# Autodesk Inventor assembly: Montagemsemfuros
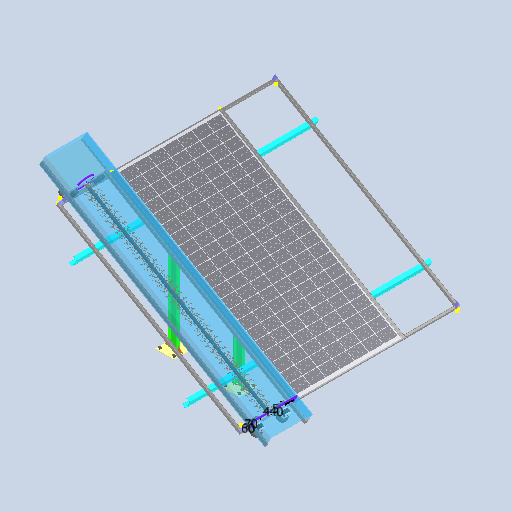
[picture p0: Inventor's stored thumbnail of the model, 512x512]
Saved by Autodesk Inventor 2025.3 (Build 293356030, 356C)
## iProperties
Created: 2019-12-15
Part Number: Montagemsemfuros
Document SubType Name: Assembly
Designer: Rubens
Sending System: SolidWorks 2021
Last Author: Mohsen
Last Saved: 2022-08-25
Author: Rubens
## Documents named in this file (36)
- C:\Users\Rubens\Downloads\Estrutura Placa - REV00\Solar Mounting Structure\Main_Solar_Structure\Main_Solar_Structure\Montagemsemfuros.iam
- C:\Users\Rubens\Downloads\Estrutura Placa - REV00\Solar Mounting Structure\Main_Solar_Structure\Main_Solar_Structure\Small_Column.ipt
- C:\Users\Rubens\Downloads\Estrutura Placa - REV00\Solar Mounting Structure\Main_Solar_Structure\Main_Solar_Structure\Large_Column.ipt
- C:\Users\Rubens\Downloads\Estrutura Placa - REV00\Solar Mounting Structure\Main_Solar_Structure\Main_Solar_Structure\Bottom_Beam.ipt
- C:\Users\Rubens\Downloads\Estrutura Placa - REV00\Solar Mounting Structure\Main_Solar_Structure\Main_Solar_Structure\Base_Plate.ipt
- C:\Users\Rubens\Downloads\Estrutura Placa - REV00\Solar Mounting Structure\Main_Solar_Structure\Main_Solar_Structure\Base_Support.ipt
- C:\Users\Rubens\Downloads\Estrutura Placa - REV00\Solar Mounting Structure\Main_Solar_Structure\Main_Solar_Structure\Beam_Support.ipt
- C:\Users\Rubens\Downloads\Estrutura Placa - REV00\Solar Mounting Structure\Main_Solar_Structure\Main_Solar_Structure\M10_Screw&Nut.iam
- C:\Users\Rubens\Downloads\Estrutura Placa - REV00\Solar Mounting Structure\Main_Solar_Structure\Main_Solar_Structure\Base.ipt
- C:\Users\Rubens\Downloads\Estrutura Placa - REV00\Solar Mounting Structure\Main_Solar_Structure\Main_Solar_Structure\ISO - 4034 - M16 - S_.ipt
- C:\Users\Rubens\Downloads\Estrutura Placa - REV00\Solar Mounting Structure\Main_Solar_Structure\Main_Solar_Structure\Base_MIR.ipt
- C:\Users\Rubens\Downloads\Estrutura Placa - REV00\Solar Mounting Structure\Main_Solar_Structure\Main_Solar_Structure\Base_Plate_MIR.ipt
- C:\Users\Rubens\Downloads\Estrutura Placa - REV00\Solar Mounting Structure\Main_Solar_Structure\Main_Solar_Structure\Base_Support_MIR.ipt
- C:\Users\Rubens\Downloads\Estrutura Placa - REV00\Solar Mounting Structure\Main_Solar_Structure\Main_Solar_Structure\Base_MIR1.ipt
- C:\Users\Rubens\Downloads\Estrutura Placa - REV00\Solar Mounting Structure\Main_Solar_Structure\Main_Solar_Structure\ISO - 4034 - M16 - S__MIR.ipt
- C:\Users\Rubens\Downloads\Estrutura Placa - REV00\Solar Mounting Structure\Main_Solar_Structure\Main_Solar_Structure\Base_MIR_MIR.ipt
- C:\Users\Rubens\Downloads\Estrutura Placa - REV00\Solar Mounting Structure\Main_Solar_Structure\Main_Solar_Structure\Top_Beam_2780.ipt
- C:\Users\Rubens\Downloads\Estrutura Placa - REV00\Solar Mounting Structure\Main_Solar_Structure\Main_Solar_Structure\Beam_Support_MIR.ipt
- C:\Users\Rubens\Downloads\Estrutura Placa - REV00\Solar Mounting Structure\Main_Solar_Structure\Main_Solar_Structure\SolarPV.ipt
- C:\Users\Rubens\Downloads\Estrutura Placa - REV00\Solar Mounting Structure\Main_Solar_Structure\Main_Solar_Structure\Perfil tubo - 30x30x3.ipt
- C:\Users\Rubens\Downloads\Estrutura Placa - REV00\Solar Mounting Structure\Main_Solar_Structure\Main_Solar_Structure\tubo 30 x 30 x 3  - 500.ipt
- C:\Users\Rubens\Downloads\Estrutura Placa - REV00\Solar Mounting Structure\Main_Solar_Structure\Main_Solar_Structure\Limitador.ipt
- C:\Users\Rubens\Downloads\Estrutura Placa - REV00\Solar Mounting Structure\Main_Solar_Structure\Main_Solar_Structure\Small_Column_MIR2.ipt
- C:\Users\Rubens\Downloads\Estrutura Placa - REV00\Solar Mounting Structure\Main_Solar_Structure\Main_Solar_Structure\Bottom_Beam_MIR2.ipt
- C:\Users\Rubens\Downloads\Estrutura Placa - REV00\Solar Mounting Structure\Main_Solar_Structure\Main_Solar_Structure\Base_Plate_MIR3.ipt
- C:\Users\Rubens\Downloads\Estrutura Placa - REV00\Solar Mounting Structure\Main_Solar_Structure\Main_Solar_Structure\Base_Support_MIR3.ipt
- C:\Users\Rubens\Downloads\Estrutura Placa - REV00\Solar Mounting Structure\Main_Solar_Structure\Main_Solar_Structure\M10_Screw&Nut_MIR1.iam
- C:\Users\Rubens\Downloads\Estrutura Placa - REV00\Solar Mounting Structure\Main_Solar_Structure\Main_Solar_Structure\ISO - 4034 - M16 - S__MIR1.ipt
- C:\Users\Rubens\Downloads\Estrutura Placa - REV00\Solar Mounting Structure\Main_Solar_Structure\Main_Solar_Structure\Base_Plate_MIR_MIR2.ipt
- C:\Users\Rubens\Downloads\Estrutura Placa - REV00\Solar Mounting Structure\Main_Solar_Structure\Main_Solar_Structure\Base_Support_MIR_MIR1.ipt
- C:\Users\Rubens\Downloads\Estrutura Placa - REV00\Solar Mounting Structure\Main_Solar_Structure\Main_Solar_Structure\ISO - 4034 - M16 - S__MIR_MIR1.ipt
- C:\Users\Rubens\Downloads\Estrutura Placa - REV00\Solar Mounting Structure\Main_Solar_Structure\Main_Solar_Structure\Large_Column_MIR3.ipt
- C:\Users\Rubens\Documents\Inventor\Content Center Files\R2025\pt-BR\ANSI B18.3.1M(5)\ANSI B18.3.1M - M8x1,25 x 20(3).ipt
- C:\Users\Rubens\Documents\Inventor\Content Center Files\R2025\pt-BR\ISO 4032(2)\ISO 4032 - M8 - ISO.ipt
- C:\Users\Rubens\Documents\Inventor\Content Center Files\R2025\pt-BR\ANSI B18.3.1M(6)\ANSI B18.3.1M - M8x1,25 x 40(1).ipt
- C:\Users\Rubens\Downloads\Limpador\MontagemREV0.iam
## Components (92 placed, 35 different names)
1. Small_Column:1 — Alinhado:6, Coincidente:67
2. Bottom_Beam:1 — Coincidente:3, Coincidente:5, Coincidente:6, Coincidente:8, Coincidente:20, Coincidente:21, Coincidente:66, Alinhado:15, Coincidente:72, Ângulo:1
3. Base_Plate:1 — Alinhado:14
4. Base_Support:1
5. Base_Support:2
6. Base_Support:3
7. Beam_Support:3 — Coincidente:3, Coincidente:5, Coincidente:23
8. Beam_Support:4 — Coincidente:6, Coincidente:8, Coincidente:22
9. M10_Screw&Nut:2 [sub-assembly]
10. M10_Screw&Nut:7 [sub-assembly]
11. M10_Screw&Nut:8 [sub-assembly]
12. M10_Screw&Nut:9 [sub-assembly]
13. M10_Screw&Nut:90 [sub-assembly]
14. M10_Screw&Nut:91 [sub-assembly]
15. Base:2
16. ISO - 4034 - M16 - S_:43
17. ISO - 4034 - M16 - S_:47
18. ISO - 4034 - M16 - S_:51
19. ISO - 4034 - M16 - S_:55
20. Base_MIR:1
21. Base_Plate_MIR:1 — Alinhado:14, Coincidente:65
22. Base_Support_MIR:1
23. Base_Support_MIR:2
24. Base_Support_MIR:3
25. Base_MIR1:1
26. ISO - 4034 - M16 - S__MIR:1
27. ISO - 4034 - M16 - S__MIR:2
28. ISO - 4034 - M16 - S__MIR:3
29. Base_MIR_MIR:1
30. Top_Beam_2780:1 — Coincidente:21, Coincidente:22, Alinhado:7, Coincidente:46, Coincidente:47, Coincidente:70, Alinhado:15, Coincidente:104
31. Top_Beam_2780:2 — Coincidente:20, Coincidente:23, Alinhado:7, Coincidente:24
32. Beam_Support_MIR:1
33. Beam_Support_MIR:2 — Coincidente:70
34. SolarPV:1 — Coincidente:24, Coincidente:48, Coincidente:49, Coincidente:50, Coincidente:55, Alinhado:22, Coincidente:113
35. Perfil tubo - 30x30x3:1 — Coincidente:46, Coincidente:48, Coincidente:52, Coincidente:53, Alinhado:9, Alinhado:10, Coincidente:55, Coincidente:57, Alinhado:12, Coincidente:108, Coincidente:109, Coincidente:110, Coincidente:111, Coincidente:114
36. Perfil tubo - 30x30x3:2 — Coincidente:47, Coincidente:54, Alinhado:11, Coincidente:56, Coincidente:105, Coincidente:106, Coincidente:107
37. Perfil tubo - 30x30x3:3 — Coincidente:49, Coincidente:50, Coincidente:79, Alinhado:20, Alinhado:21, Alinhado:22, Alinhado:23
38. tubo 30 x 30 x 3  - 500:1 — Coincidente:53, Alinhado:9, Alinhado:10, Coincidente:54, Alinhado:11, Coincidente:56, Coincidente:82, Alinhado:26
39. tubo 30 x 30 x 3  - 500:2 — Coincidente:52, Coincidente:57, Alinhado:12, Coincidente:81, Coincidente:112, Alinhado:27
40. Perfil tubo - 30x30x3:4 — Coincidente:58, Alinhado:13, Coincidente:59, Coincidente:80, Coincidente:83, Alinhado:19, Coincidente:84, Coincidente:85, Coincidente:100, Coincidente:101
41. tubo 30 x 30 x 3  - 500:3 — Coincidente:58, Alinhado:13, Coincidente:59, Alinhado:21
42. tubo 30 x 30 x 3  - 500:4 — Coincidente:79, Coincidente:80, Alinhado:19, Alinhado:20, Alinhado:23
43. ISO - 4034 - M16 - S__MIR:4 — Coincidente:65
44. Large_Column:1 — Coincidente:66, Coincidente:67, Coincidente:86, Coincidente:87, Coincidente:88, Coincidente:89
45. Limitador:1 — Coincidente:83
46. Limitador:2 — Coincidente:81
47. Limitador:3 — Coincidente:82
48. Limitador:4 — Coincidente:84, Coincidente:85
49. M10_Screw&Nut:92 [sub-assembly] — Coincidente:86
50. M10_Screw&Nut:93 [sub-assembly] — Coincidente:88
51. M10_Screw&Nut:94 [sub-assembly] — Coincidente:89
52. M10_Screw&Nut:96 [sub-assembly] — Coincidente:87
53. Small_Column_MIR2:1 — Alinhado:24, Coincidente:91
54. Bottom_Beam_MIR2:1 — Coincidente:92, Ângulo:2, Coincidente:93
55. Base_Plate_MIR3:1 — Alinhado:25
56. Base_Support_MIR3:1
57. Base_Support_MIR3:2
58. Base_Support_MIR3:3
59. M10_Screw&Nut_MIR1:1 [sub-assembly]
60. M10_Screw&Nut_MIR1:2 [sub-assembly]
61. M10_Screw&Nut_MIR1:3 [sub-assembly]
62. M10_Screw&Nut_MIR1:4 [sub-assembly]
63. ISO - 4034 - M16 - S__MIR1:1
64. ISO - 4034 - M16 - S__MIR1:2
65. ISO - 4034 - M16 - S__MIR1:3
66. ISO - 4034 - M16 - S__MIR1:4
67. Base_Plate_MIR_MIR2:1 — Alinhado:25, Coincidente:90
68. Base_Support_MIR_MIR1:1
69. Base_Support_MIR_MIR1:2
70. Base_Support_MIR_MIR1:3
71. ISO - 4034 - M16 - S__MIR_MIR1:1
72. ISO - 4034 - M16 - S__MIR_MIR1:2
73. ISO - 4034 - M16 - S__MIR_MIR1:3
74. ISO - 4034 - M16 - S__MIR_MIR1:4 — Coincidente:90
75. Large_Column_MIR3:1 — Coincidente:91, Coincidente:92, Coincidente:94, Coincidente:95, Coincidente:96, Coincidente:97
76. M10_Screw&Nut_MIR1:5 [sub-assembly] — Coincidente:94
77. M10_Screw&Nut_MIR1:6 [sub-assembly] — Coincidente:95
78. M10_Screw&Nut_MIR1:7 [sub-assembly] — Coincidente:96
79. M10_Screw&Nut_MIR1:8 [sub-assembly] — Coincidente:97
80. Parafuso Allen de cabeça forjada e furada - 6 furos - Métrica M8x1,25 x 20:1
81. ISO 4032 M8:1 — Coincidente:100
82. ISO 4032 M8:2 — Coincidente:101
83. Parafuso Allen de cabeça forjado - Métrica M8x1,25 x 40:3 — Coincidente:106
84. ISO 4032 M8:3 — Coincidente:107
85. Parafuso Allen de cabeça forjado - Métrica M8x1,25 x 40:4 — Coincidente:104
86. ISO 4032 M8:4 — Coincidente:105
87. Parafuso Allen de cabeça forjado - Métrica M8x1,25 x 40:5 — Coincidente:108
88. Parafuso Allen de cabeça forjado - Métrica M8x1,25 x 40:6 — Coincidente:109
89. ISO 4032 M8:5 — Coincidente:110
90. ISO 4032 M8:6 — Coincidente:111
91. MontagemREV0:2 [sub-assembly] — Coincidente:112, Alinhado:26, Coincidente:113
92. SolarPV:2 — Alinhado:27, Coincidente:114
## Relationships (82: Mate 61, Flush 19, Angle 2)
- Coincidente:3 [Mate]: Bottom_Beam:1 ↔ Beam_Support:3
- Coincidente:5 [Mate]: Bottom_Beam:1 ↔ Beam_Support:3
- Coincidente:6 [Mate]: Bottom_Beam:1 ↔ Beam_Support:4
- Coincidente:8 [Mate]: Bottom_Beam:1 ↔ Beam_Support:4
- Alinhado:6 [Flush] (300 mm): Small_Column:1
- Coincidente:20 [Mate]: Bottom_Beam:1 ↔ Top_Beam_2780:2
- Coincidente:21 [Mate]: Bottom_Beam:1 ↔ Top_Beam_2780:1
- Coincidente:22 [Mate]: Beam_Support:4 ↔ Top_Beam_2780:1
- Coincidente:23 [Mate]: Beam_Support:3 ↔ Top_Beam_2780:2
- Alinhado:7 [Flush]: Top_Beam_2780:1 ↔ Top_Beam_2780:2
- Coincidente:24 [Mate]: Top_Beam_2780:2 ↔ SolarPV:1
- Coincidente:46 [Mate]: Top_Beam_2780:1 ↔ Perfil tubo - 30x30x3:1
- Coincidente:47 [Mate]: Top_Beam_2780:1 ↔ Perfil tubo - 30x30x3:2
- Coincidente:48 [Mate]: SolarPV:1 ↔ Perfil tubo - 30x30x3:1
- Coincidente:49 [Mate]: SolarPV:1 ↔ Perfil tubo - 30x30x3:3
- Coincidente:50 [Mate]: SolarPV:1 ↔ Perfil tubo - 30x30x3:3
- Coincidente:52 [Mate]: Perfil tubo - 30x30x3:1 ↔ tubo 30 x 30 x 3  - 500:2
- Coincidente:53 [Mate]: Perfil tubo - 30x30x3:1 ↔ tubo 30 x 30 x 3  - 500:1
- Alinhado:9 [Flush]: Perfil tubo - 30x30x3:1 ↔ tubo 30 x 30 x 3  - 500:1
- Alinhado:10 [Flush]: Perfil tubo - 30x30x3:1 ↔ tubo 30 x 30 x 3  - 500:1
- Coincidente:54 [Mate]: Perfil tubo - 30x30x3:2 ↔ tubo 30 x 30 x 3  - 500:1
- Alinhado:11 [Flush]: Perfil tubo - 30x30x3:2 ↔ tubo 30 x 30 x 3  - 500:1
- Coincidente:55 [Mate]: SolarPV:1 ↔ Perfil tubo - 30x30x3:1
- Coincidente:56 [Mate]: Perfil tubo - 30x30x3:2 ↔ tubo 30 x 30 x 3  - 500:1
- Coincidente:57 [Mate]: Perfil tubo - 30x30x3:1 ↔ tubo 30 x 30 x 3  - 500:2
- Alinhado:12 [Flush]: Perfil tubo - 30x30x3:1 ↔ tubo 30 x 30 x 3  - 500:2
- Coincidente:58 [Mate]: Perfil tubo - 30x30x3:4 ↔ tubo 30 x 30 x 3  - 500:3
- Alinhado:13 [Flush]: Perfil tubo - 30x30x3:4 ↔ tubo 30 x 30 x 3  - 500:3
- Coincidente:59 [Mate]: Perfil tubo - 30x30x3:4 ↔ tubo 30 x 30 x 3  - 500:3
- Alinhado:14 [Flush]: Base_Plate:1 ↔ Base_Plate_MIR:1
- Coincidente:65 [Mate]: Base_Plate_MIR:1 ↔ ISO - 4034 - M16 - S__MIR:4
- Coincidente:66 [Mate]: Bottom_Beam:1 ↔ Large_Column:1
- Coincidente:67 [Mate] (600 mm): Small_Column:1 ↔ Large_Column:1
- Coincidente:70 [Mate]: Top_Beam_2780:1 ↔ Beam_Support_MIR:2
- Alinhado:15 [Flush] (-900 mm): Bottom_Beam:1 ↔ Top_Beam_2780:1
- Coincidente:72 [Mate]: Bottom_Beam:1
- Ângulo:1 [Angle] (0 deg): Bottom_Beam:1
- Alinhado:16 [Flush] (-450 mm)
- Coincidente:79 [Mate]: Perfil tubo - 30x30x3:3 ↔ tubo 30 x 30 x 3  - 500:4
- Coincidente:80 [Mate]: Perfil tubo - 30x30x3:4 ↔ tubo 30 x 30 x 3  - 500:4
- Coincidente:81 [Mate]: tubo 30 x 30 x 3  - 500:2 ↔ Limitador:2
- Coincidente:82 [Mate]: tubo 30 x 30 x 3  - 500:1 ↔ Limitador:3
- Coincidente:83 [Mate]: Perfil tubo - 30x30x3:4 ↔ Limitador:1
- Alinhado:19 [Flush]: Perfil tubo - 30x30x3:4 ↔ tubo 30 x 30 x 3  - 500:4
- Alinhado:20 [Flush]: Perfil tubo - 30x30x3:3 ↔ tubo 30 x 30 x 3  - 500:4
- Coincidente:84 [Mate]: Perfil tubo - 30x30x3:4 ↔ Limitador:4
- Coincidente:85 [Mate]: Perfil tubo - 30x30x3:4 ↔ Limitador:4
- Alinhado:21 [Flush]: Perfil tubo - 30x30x3:3 ↔ tubo 30 x 30 x 3  - 500:3
- Alinhado:22 [Flush]: SolarPV:1 ↔ Perfil tubo - 30x30x3:3
- Alinhado:23 [Flush]: Perfil tubo - 30x30x3:3 ↔ tubo 30 x 30 x 3  - 500:4
- Coincidente:86 [Mate]: Large_Column:1 ↔ M10_Screw&Nut:92
- Coincidente:87 [Mate]: Large_Column:1 ↔ M10_Screw&Nut:96
- Coincidente:88 [Mate]: Large_Column:1 ↔ M10_Screw&Nut:93
- Coincidente:89 [Mate]: Large_Column:1 ↔ M10_Screw&Nut:94
- Alinhado:24 [Flush] (300 mm): Small_Column_MIR2:1
- Alinhado:25 [Flush]: Base_Plate_MIR3:1 ↔ Base_Plate_MIR_MIR2:1
- Coincidente:90 [Mate]: Base_Plate_MIR_MIR2:1 ↔ ISO - 4034 - M16 - S__MIR_MIR1:4
- Coincidente:91 [Mate] (600 mm): Small_Column_MIR2:1 ↔ Large_Column_MIR3:1
- Coincidente:92 [Mate]: Bottom_Beam_MIR2:1 ↔ Large_Column_MIR3:1
- Ângulo:2 [Angle] (0 deg): Bottom_Beam_MIR2:1
- Coincidente:93 [Mate]: Bottom_Beam_MIR2:1
- Coincidente:94 [Mate]: Large_Column_MIR3:1 ↔ M10_Screw&Nut_MIR1:5
- Coincidente:95 [Mate]: Large_Column_MIR3:1 ↔ M10_Screw&Nut_MIR1:6
- Coincidente:96 [Mate]: Large_Column_MIR3:1 ↔ M10_Screw&Nut_MIR1:7
- Coincidente:97 [Mate]: Large_Column_MIR3:1 ↔ M10_Screw&Nut_MIR1:8
- Coincidente:100 [Mate]: Perfil tubo - 30x30x3:4 ↔ ISO 4032 M8:1
- Coincidente:101 [Mate]: Perfil tubo - 30x30x3:4 ↔ ISO 4032 M8:2
- [Mate]: Parafuso Allen de cabeça forjado - Métrica M8x1,25 x 40:3 ↔ ISO 4032 M8:3
- [Mate]: Parafuso Allen de cabeça forjado - Métrica M8x1,25 x 40:4 ↔ ISO 4032 M8:4
- Coincidente:104 [Mate]: Top_Beam_2780:1 ↔ Parafuso Allen de cabeça forjado - Métrica M8x1,25 x 40:4
- Coincidente:105 [Mate]: Perfil tubo - 30x30x3:2 ↔ ISO 4032 M8:4
- Coincidente:106 [Mate]: Perfil tubo - 30x30x3:2 ↔ Parafuso Allen de cabeça forjado - Métrica M8x1,25 x 40:3
- Coincidente:107 [Mate]: Perfil tubo - 30x30x3:2 ↔ ISO 4032 M8:3
- Coincidente:108 [Mate]: Perfil tubo - 30x30x3:1 ↔ Parafuso Allen de cabeça forjado - Métrica M8x1,25 x 40:5
- Coincidente:109 [Mate]: Perfil tubo - 30x30x3:1 ↔ Parafuso Allen de cabeça forjado - Métrica M8x1,25 x 40:6
- Coincidente:110 [Mate]: Perfil tubo - 30x30x3:1 ↔ ISO 4032 M8:5
- Coincidente:111 [Mate]: Perfil tubo - 30x30x3:1 ↔ ISO 4032 M8:6
- Coincidente:112 [Mate] (50 mm): tubo 30 x 30 x 3  - 500:2 ↔ MontagemREV0:2
- Alinhado:26 [Flush] (15 mm): tubo 30 x 30 x 3  - 500:1 ↔ MontagemREV0:2
- Coincidente:113 [Mate] (50 mm): SolarPV:1 ↔ MontagemREV0:2
- Alinhado:27 [Flush]: tubo 30 x 30 x 3  - 500:2 ↔ SolarPV:2
- Coincidente:114 [Mate]: Perfil tubo - 30x30x3:1 ↔ SolarPV:2
## Named parameters: d149_d146 = 0 mm, d150_d146 = 0 mm
